# Autodesk Inventor assembly: OneRobotAssembly
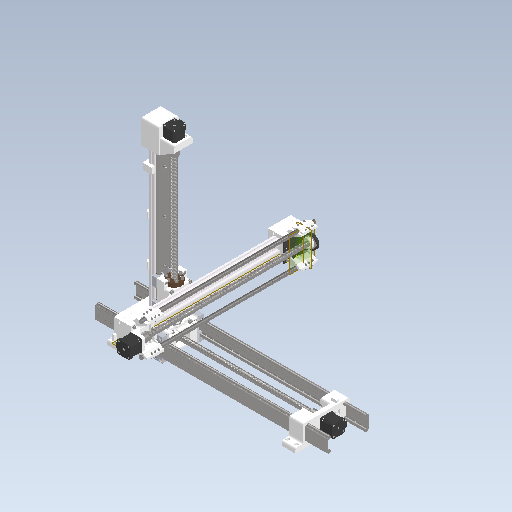
[picture p0: Inventor's stored thumbnail of the model, 512x512]
Saved by Autodesk Inventor 2020 (Build 240168000, 168)
## iProperties
Created: 2022-06-28
Part Number: OneRobotAssembly
Document SubType Name: Assembly
Designer: mikoma
Author: mikoma
## Documents named in this file (4)
- D:\MGR\model\Workspaces\Obszar roboczy\assembly_v3\OneRobotAssembly.iam
- D:\MGR\model\Workspaces\Obszar roboczy\assembly_v3\Z\Z.iam
- D:\MGR\model\Workspaces\Obszar roboczy\assembly_v3\X\X.iam
- D:\MGR\model\Workspaces\Obszar roboczy\assembly_v3\Y\Y.iam
## Components (3 placed, 3 different names)
1. Z:1 [sub-assembly] — Zestawiające:5, Zestawiające:6
2. X:1 [sub-assembly] — Zestawiające:5
3. Y:1 [sub-assembly] — Zestawiające:6
## Relationships (6: Mate 6)
- [Mate]: Z:1 ↔ Y:1
- [Mate]: Z:1 ↔ Y:1
- [Mate]: Z:1 ↔ X:1
- [Mate]: Z:1 ↔ X:1
- Zestawiające:5 [Mate]: Z:1 ↔ X:1
- Zestawiające:6 [Mate]: Z:1 ↔ Y:1
